# Autodesk Inventor assembly: P80 Gearbox 3-stage
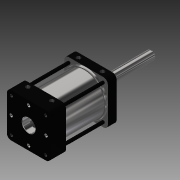
[picture p0: Inventor's stored thumbnail of the model, 180x180]
Saved by Autodesk Inventor 2013 (Build 170138000, 138)
## iProperties
Created: 2013-02-10
Part Number: P80 Gearbox 3-stage
Document SubType Name: Assembly
Designer: Moses
Mass: 1562.8 g
Surface Area: 700.255 cm^2
Volume: 199.083 cm^3
Density: 7.85 g/cm^3
Author: Moses
## Documents named in this file (7)
- C:\Users\Moses\Documents\GitHub\frc2013CAD\Cimber actual\P80 Gearbox\P80 Gearbox 3-stage.iam
- C:\Users\Moses\Documents\GitHub\frc2013CAD\Cimber actual\P80 Gearbox\P80 Front Block.ipt
- C:\Users\Moses\Documents\GitHub\frc2013CAD\Cimber actual\P80 Gearbox\Ball Bearing 12x28x8.ipt
- C:\Users\Moses\Documents\GitHub\frc2013CAD\Cimber actual\P80 Gearbox\91290A192\91290A192.ipt
- C:\Users\Moses\Documents\GitHub\frc2013CAD\Cimber actual\P80 Gearbox\P80 Ring Gear 3-stage.ipt
- C:\Users\Moses\Documents\GitHub\frc2013CAD\Cimber actual\P80 Gearbox\P80 Motor Block.ipt
- C:\Users\Moses\Documents\GitHub\frc2013CAD\Cimber actual\P80 Gearbox\P80 Shaft (3.25 inch).ipt
## Components (10 placed, 6 different names)
1. P80 Front Block:1 — Insert:1, Insert:2, Insert:3, Insert:4, Insert:5, Insert:6, Insert:7, Insert:9
2. Ball Bearing 12x28x8:1 — Insert:1
3. 91290A192:1 — Insert:3
4. 91290A192:2 — Insert:2
5. 91290A192:3 — Insert:5
6. 91290A192:4 — Insert:4, Mate:1
7. P80 Ring Gear 3-stage:1 — Insert:6, Insert:8
8. Ball Bearing 12x28x8:2 — Insert:7
9. P80 Motor Block:1 — Insert:8, Mate:1
10. P80 Shaft (3.25 inch):1 — Insert:9
## Relationships (10: Insert 9, Mate 1)
- Insert:1 (0.254 mm): P80 Front Block:1 ↔ Ball Bearing 12x28x8:1
- Insert:2: P80 Front Block:1 ↔ 91290A192:2
- Insert:3: P80 Front Block:1 ↔ 91290A192:1
- Insert:4: P80 Front Block:1 ↔ 91290A192:4
- Insert:5: P80 Front Block:1 ↔ 91290A192:3
- Insert:6: P80 Front Block:1 ↔ P80 Ring Gear 3-stage:1
- Insert:7 (0.254 mm): P80 Front Block:1 ↔ Ball Bearing 12x28x8:2
- Insert:8: P80 Ring Gear 3-stage:1 ↔ P80 Motor Block:1
- Mate:1: 91290A192:4 ↔ P80 Motor Block:1
- Insert:9: P80 Front Block:1 ↔ P80 Shaft (3.25 inch):1
